# Autodesk Inventor assembly: enc - FrontPanel Oben V2 - Assembly
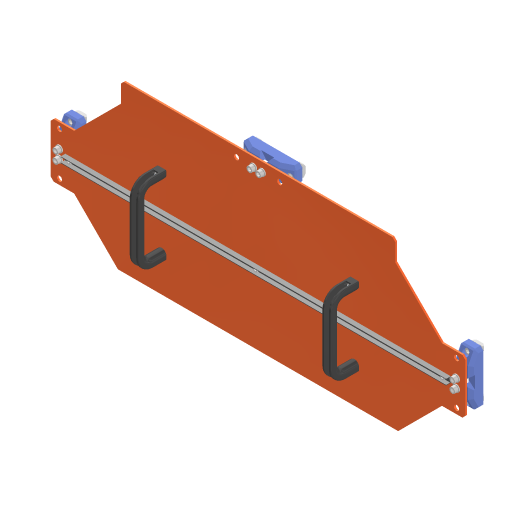
[picture p0: Inventor's stored thumbnail of the model, 512x512]
Saved by Autodesk Inventor 2023.2 (Build 272271000, 271)
## iProperties
Created: 2023-12-14
Part Number: enc - FrontPanel Oben V2 - Assembly
Document SubType Name: Assembly
Designer: Nils Bade
Author: Nils Bade
## Documents named in this file (7)
- C:\Users\nilsb\Documents\Inventor\Projektarbeit-Bade\Enclosure\enc - FrontPanel Oben V2 - Assembly.iam
- C:\Users\nilsb\Documents\Inventor\Projektarbeit-Bade\Enclosure\Magnet PanelFrame Straight connected.iam
- C:\Users\nilsb\Documents\Inventor\Projektarbeit-Bade\Enclosure\U-Profil PanelSupport 10x8x660mm.ipt
- C:\Users\nilsb\Documents\Inventor\Projektarbeit-Bade\Schrauben\Cap Head Screw M4x8 - DIN912.ipt
- C:\Users\nilsb\Documents\Inventor\Projektarbeit-Bade\RatRig_Standards\Hex Nut - M4 DIN934.ipt
- C:\Users\nilsb\Documents\Inventor\Projektarbeit-Bade\Enclosure\enc - FrontPanel Oben V2.ipt
- C:\Users\nilsb\Documents\Inventor\Projektarbeit-Bade\Enclosure\item_Handgriff_PA120_Assembly.iam
## Components (13 placed, 6 different names)
1. Magnet PanelFrame Straight connected:1 [sub-assembly]
2. Magnet PanelFrame Straight connected:2 [sub-assembly]
3. Magnet PanelFrame Straight connected:3 [sub-assembly]
4. item_Handgriff_120er:1 [sub-assembly] — Passend:55, Passend:57, Passend:60
5. item_Handgriff_120er:2 [sub-assembly] — Passend:56, Passend:58, Passend:59
6. U-Profil PanelSupport 10x8x265mm:1 — Passend:47, Passend:48, Passend:49, Passend:50, Passend:53, Passend:54
7. Hex Nut - M4 DIN934:3 — Passend:21
8. Hex Nut - M4 DIN934:2 — Passend:20
9. Hex Nut - M4 DIN934:1 — Passend:19
10. Cap Head Screw M4x8 - DIN912:3 — Passend:19, Passend:52, Passend:54
11. Cap Head Screw M4x8 - DIN912:2 — Passend:20, Passend:50
12. Cap Head Screw M4x8 - DIN912:1 — Passend:21, Passend:51, Passend:53
13. enc - FrontPanel Oben V2 - 295x720:2 — Passend:47, Passend:48, Passend:49, Passend:51, Passend:52, Passend:55, Passend:56, Passend:57, Passend:58, Passend:59, Passend:60
## Relationships (30: Mate 30)
- [Mate]: Magnet PanelFrame Straight connected:3 ↔ enc - FrontPanel Oben V2 - 295x720:2
- [Mate]: Magnet PanelFrame Straight connected:3 ↔ enc - FrontPanel Oben V2 - 295x720:2
- [Mate]: Magnet PanelFrame Straight connected:3 ↔ enc - FrontPanel Oben V2 - 295x720:2
- [Mate]: Magnet PanelFrame Straight connected:1 ↔ enc - FrontPanel Oben V2 - 295x720:2
- [Mate]: Magnet PanelFrame Straight connected:1 ↔ enc - FrontPanel Oben V2 - 295x720:2
- [Mate]: Magnet PanelFrame Straight connected:1 ↔ enc - FrontPanel Oben V2 - 295x720:2
- [Mate]: Magnet PanelFrame Straight connected:2 ↔ enc - FrontPanel Oben V2 - 295x720:2
- [Mate]: Magnet PanelFrame Straight connected:2 ↔ enc - FrontPanel Oben V2 - 295x720:2
- [Mate]: Magnet PanelFrame Straight connected:2 ↔ enc - FrontPanel Oben V2 - 295x720:2
- [Mate]: Cap Head Screw M4x8 - DIN912:2 ↔ enc - FrontPanel Oben V2 - 295x720:2
- Passend:19 [Mate]: Hex Nut - M4 DIN934:1 ↔ Cap Head Screw M4x8 - DIN912:3
- Passend:20 [Mate]: Hex Nut - M4 DIN934:2 ↔ Cap Head Screw M4x8 - DIN912:2
- Passend:21 [Mate]: Hex Nut - M4 DIN934:3 ↔ Cap Head Screw M4x8 - DIN912:1
- [Mate]: Hex Nut - M4 DIN934:1 ↔ enc - FrontPanel Oben V2 - 295x720:2
- [Mate]: Hex Nut - M4 DIN934:2 ↔ enc - FrontPanel Oben V2 - 295x720:2
- [Mate]: Hex Nut - M4 DIN934:3 ↔ enc - FrontPanel Oben V2 - 295x720:2
- Passend:47 [Mate]: U-Profil PanelSupport 10x8x265mm:1 ↔ enc - FrontPanel Oben V2 - 295x720:2
- Passend:48 [Mate]: U-Profil PanelSupport 10x8x265mm:1 ↔ enc - FrontPanel Oben V2 - 295x720:2
- Passend:49 [Mate]: U-Profil PanelSupport 10x8x265mm:1 ↔ enc - FrontPanel Oben V2 - 295x720:2
- Passend:50 [Mate]: U-Profil PanelSupport 10x8x265mm:1 ↔ Cap Head Screw M4x8 - DIN912:2
- Passend:51 [Mate]: Cap Head Screw M4x8 - DIN912:1 ↔ enc - FrontPanel Oben V2 - 295x720:2
- Passend:52 [Mate]: Cap Head Screw M4x8 - DIN912:3 ↔ enc - FrontPanel Oben V2 - 295x720:2
- Passend:53 [Mate]: U-Profil PanelSupport 10x8x265mm:1 ↔ Cap Head Screw M4x8 - DIN912:1
- Passend:54 [Mate]: U-Profil PanelSupport 10x8x265mm:1 ↔ Cap Head Screw M4x8 - DIN912:3
- Passend:55 [Mate]: item_Handgriff_120er:1 ↔ enc - FrontPanel Oben V2 - 295x720:2
- Passend:56 [Mate]: item_Handgriff_120er:2 ↔ enc - FrontPanel Oben V2 - 295x720:2
- Passend:57 [Mate]: item_Handgriff_120er:1 ↔ enc - FrontPanel Oben V2 - 295x720:2
- Passend:58 [Mate]: item_Handgriff_120er:2 ↔ enc - FrontPanel Oben V2 - 295x720:2
- Passend:59 [Mate]: item_Handgriff_120er:2 ↔ enc - FrontPanel Oben V2 - 295x720:2
- Passend:60 [Mate]: item_Handgriff_120er:1 ↔ enc - FrontPanel Oben V2 - 295x720:2
